# Autodesk Inventor assembly: motor w-screw
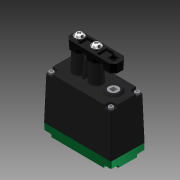
[picture p0: Inventor's stored thumbnail of the model, 180x180]
Saved by Autodesk Inventor 2014 (Build 180170000, 170)
## iProperties
Created: 2014-08-19
Part Number: motor w-screw
Document SubType Name: Assembly
Designer: Josef
Author: Josef
## Documents named in this file (4)
- C:\Users\Josef\Documents\Vex parts\motor w-screw.iam
- C:\Users\Josef\Documents\Vex parts\motors\393 motor.iam
- C:\Users\Josef\Documents\Vex parts\Other Parts\Bearing Flat, Delrin.ipt
- C:\Users\Josef\Documents\Vex parts\Screws & Nuts\Screw 6-32 x 0.500''-Silver.ipt
## Components (4 placed, 3 different names)
1. 393 motor:1 [sub-assembly] — Mate:1, Mate:2, Mate:3
2. Bearing Flat, Delrin:1 — Mate:1, Mate:2, Mate:3, Mate:5, Mate:6
3. Screw 6-32 x 0.500''-Silver:1 — Mate:5
4. Screw 6-32 x 0.500''-Silver:2 — Mate:6
## Relationships (5: Mate 5)
- Mate:1: 393 motor:1 ↔ Bearing Flat, Delrin:1
- Mate:2: 393 motor:1 ↔ Bearing Flat, Delrin:1
- Mate:3: 393 motor:1 ↔ Bearing Flat, Delrin:1
- Mate:5: Bearing Flat, Delrin:1 ↔ Screw 6-32 x 0.500''-Silver:1
- Mate:6: Bearing Flat, Delrin:1 ↔ Screw 6-32 x 0.500''-Silver:2
